# Autodesk Inventor assembly: sample complete assembly
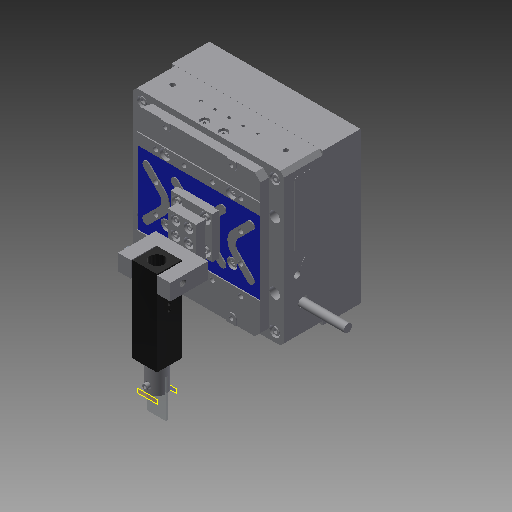
[picture p0: Inventor's stored thumbnail of the model, 512x512]
Saved by Autodesk Inventor 2019 (Build 230136000, 136)
## iProperties
Created: 2019-03-15
Part Number: sample complete assembly
Document SubType Name: Assembly
Designer: Saumya
Author: Saumya
## Documents named in this file (12)
- C:\Users\Saumya\Documents\Inventor\ClearedTissue\clear tissue_2_cad\ClearedTissueMicroscope_CAD\clear tissue assembly\Parts\sample complete assembly.iam
- C:\Users\Saumya\Documents\Inventor\ClearedTissue\clear tissue_2_cad\ClearedTissueMicroscope_CAD\clear tissue assembly\Parts\male_long_part2_9_2018.ipt
- C:\Users\Saumya\Documents\Inventor\ClearedTissue\clear tissue_2_cad\ClearedTissueMicroscope_CAD\clear tissue assembly\Parts\Sample holder long L_V4.ipt
- C:\Users\Saumya\Documents\Inventor\ClearedTissue\clear tissue_2_cad\ClearedTissueMicroscope_CAD\clear tissue assembly\Parts\sample holder mount on PI_V_522_v2.ipt
- C:\Users\Saumya\Documents\Inventor\ClearedTissue\clear tissue_2_cad\ClearedTissueMicroscope_CAD\clear tissue assembly\Parts\slit-adapter-clear-scope_8_2018.ipt
- C:\Users\Saumya\Documents\Inventor\ClearedTissue\clear tissue_2_cad\ClearedTissueMicroscope_CAD\clear tissue assembly\Parts\glass slide.ipt
- C:\Users\Saumya\Documents\Inventor\ClearedTissue\clear tissue_2_cad\ClearedTissueMicroscope_CAD\clear tissue assembly\Parts\V-522.1AA_KUNDENMODELL V-522.1AA.ipt
- C:\Users\Saumya\Documents\Inventor\ClearedTissue\clear tissue_2_cad\ClearedTissueMicroscope_CAD\clear tissue assembly\Parts\Adapter_V_522_and_Sutter_V4.0001.ipt
- C:\Users\Saumya\Documents\Inventor\ClearedTissue\clear tissue_2_cad\ClearedTissueMicroscope_CAD\clear tissue assembly\Parts\1-64 screw.ipt
- C:\Users\Saumya\Documents\Inventor\ClearedTissue\clear tissue_2_cad\ClearedTissueMicroscope_CAD\clear tissue assembly\Parts\unc 3-48 screw.ipt
- C:\Users\Saumya\Documents\Inventor\ClearedTissue\clear tissue_2_cad\ClearedTissueMicroscope_CAD\clear tissue assembly\Parts\m2.5.ipt
- C:\Users\Saumya\Documents\Inventor\ClearedTissue\clear tissue_2_cad\ClearedTissueMicroscope_CAD\clear tissue assembly\Parts\grainger-1ME94.ipt
## Components (25 placed, 11 different names)
1. male_long_part2_9_2018:1 — Cylindrical:1
2. Sample holder long L_V4:2
3. sample holder mount on PI_V_522_v2:1
4. slit-adapter-clear-scope_8_2018:1 — Cylindrical:1, Mate:1
5. glass slide:1 — Mate:1
6. Adapter_V_522_and_Sutter_V4.0001:1 — Mate:2
7. V-522.1AA_KUNDENMODELL V-522.1AA:2 — Mate:2
8. 1-64 screw:1
9. 1-64 screw:2
10. 1-64 screw:3
11. 1-64 screw:4
12. 1-64 screw:5
13. 1-64 screw:6
14. 1-64 screw:7
15. 1-64 screw:8
16. unc 3-48 screw:1
17. unc 3-48 screw:2
18. unc 3-48 screw:3
19. unc 3-48 screw:4
20. m2.5:1
21. m2.5:2
22. m2.5:3
23. m2.5:4
24. 1-64 screw:9
25. grainger-1ME94:1
## Relationships (3: Mate 2, CylindricalJoint 1)
- Cylindrical:1: male_long_part2_9_2018:1 ↔ slit-adapter-clear-scope_8_2018:1
- Mate:1: slit-adapter-clear-scope_8_2018:1 ↔ glass slide:1
- Mate:2: Adapter_V_522_and_Sutter_V4.0001:1 ↔ V-522.1AA_KUNDENMODELL V-522.1AA:2
